# Autodesk Inventor assembly: outer rails
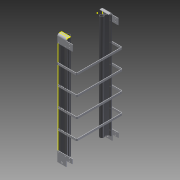
[picture p0: Inventor's stored thumbnail of the model, 180x180]
Saved by Autodesk Inventor 2013 (Build 170138000, 138)
## iProperties
Created: 2013-01-27
Part Number: outer rails
Document SubType Name: Assembly
Designer: Arpan
Author: Arpan
## Documents named in this file (6)
- C:\Users\Arpan\Documents\GitHub\frc2013CAD\Cimber actual\outer rails.iam
- C:\Users\Arpan\Documents\GitHub\frc2013CAD\Cimber actual\Shaft 26 inch.ipt
- C:\Users\Arpan\Documents\GitHub\frc2013CAD\Cimber actual\tie-together tier 2.ipt
- C:\Users\Arpan\Documents\GitHub\frc2013CAD\Cimber actual\endstop.ipt
- C:\Users\Arpan\Documents\GitHub\frc2013CAD\Cimber actual\endstop 2.ipt
- C:\Users\Arpan\Documents\GitHub\frc2013CAD\Cimber actual\arm mout.ipt
## Components (10 placed, 5 different names)
1. Shaft 26 inch:1 — Angle:1, Flush:1, Mate:5, Mate:6, Mate:7, Mate:8, Mate:9, Mate:10, Mate:11, Mate:12, Mate:14, Mate:24, Mate:25, Mate:26, Mate:30, Mate:31, Mate:32
2. Shaft 26 inch:2 — Angle:1, Flush:1, Mate:2, Angle:2, Mate:3, Mate:13, Mate:16, Mate:17, Mate:21, Mate:22, Mate:23, Flush:2, Mate:27, Mate:28, Mate:29, Mate:33
3. tie-together tier 2:1 — Mate:2, Angle:2, Mate:3, Mate:5, Mate:6, Mate:33
4. tie-together tier 2:2 — Mate:7, Mate:8, Mate:9
5. tie-together tier 2:3 — Mate:10, Mate:11, Mate:12, Mate:13
6. tie-together tier 2:4 — Mate:14, Mate:16, Mate:17
7. endstop:1 — Mate:24, Mate:25, Mate:26
8. endstop 2:1 — Mate:21, Mate:22, Mate:23
9. arm mout:2 — Flush:2, Mate:27, Mate:28, Mate:29
10. arm mout:3 — Mate:30, Mate:31, Mate:32
## Relationships (31: Mate 27, Angle 2, Flush 2)
- Angle:1 (180 deg): Shaft 26 inch:1 ↔ Shaft 26 inch:2
- Flush:1: Shaft 26 inch:1 ↔ Shaft 26 inch:2
- Mate:2: Shaft 26 inch:2 ↔ tie-together tier 2:1
- Angle:2 (0 deg): Shaft 26 inch:2 ↔ tie-together tier 2:1
- Mate:3: Shaft 26 inch:2 ↔ tie-together tier 2:1
- Mate:5: Shaft 26 inch:1 ↔ tie-together tier 2:1
- Mate:6: Shaft 26 inch:1 ↔ tie-together tier 2:1
- Mate:7: Shaft 26 inch:1 ↔ tie-together tier 2:2
- Mate:8: Shaft 26 inch:1 ↔ tie-together tier 2:2
- Mate:9: Shaft 26 inch:1 ↔ tie-together tier 2:2
- Mate:10: Shaft 26 inch:1 ↔ tie-together tier 2:3
- Mate:11: Shaft 26 inch:1 ↔ tie-together tier 2:3
- Mate:12: Shaft 26 inch:1 ↔ tie-together tier 2:3
- Mate:13: Shaft 26 inch:2 ↔ tie-together tier 2:3
- Mate:14: Shaft 26 inch:1 ↔ tie-together tier 2:4
- Mate:16: Shaft 26 inch:2 ↔ tie-together tier 2:4
- Mate:17: Shaft 26 inch:2 ↔ tie-together tier 2:4
- Mate:21: Shaft 26 inch:2 ↔ endstop 2:1
- Mate:22: Shaft 26 inch:2 ↔ endstop 2:1
- Mate:23: Shaft 26 inch:2 ↔ endstop 2:1
- Mate:24: Shaft 26 inch:1 ↔ endstop:1
- Mate:25: Shaft 26 inch:1 ↔ endstop:1
- Mate:26: Shaft 26 inch:1 ↔ endstop:1
- Flush:2: Shaft 26 inch:2 ↔ arm mout:2
- Mate:27: Shaft 26 inch:2 ↔ arm mout:2
- Mate:28: Shaft 26 inch:2 ↔ arm mout:2
- Mate:29: Shaft 26 inch:2 ↔ arm mout:2
- Mate:30: Shaft 26 inch:1 ↔ arm mout:3
- Mate:31: Shaft 26 inch:1 ↔ arm mout:3
- Mate:32: Shaft 26 inch:1 ↔ arm mout:3
- Mate:33: Shaft 26 inch:2 ↔ tie-together tier 2:1
